# Autodesk Inventor assembly: FullApparatus
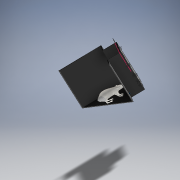
[picture p0: Inventor's stored thumbnail of the model, 180x180]
Saved by Autodesk Inventor 2020 (Build 240168000, 168)
## iProperties
Created: 2019-09-17
Part Number: FullApparatus
Document SubType Name: Assembly
Designer: Knowblesse
Author: Knowblesse
## Documents named in this file (5)
- C:\VCF\Lobster\Apparatus\FullApparatus.iam
- C:\VCF\Lobster\Apparatus\Arena\Main.ipt
- C:\VCF\Lobster\Apparatus\Robot\Motor_Panel.iam
- C:\VCF\Lobster\Apparatus\Arena\IRLight.ipt
- C:\VCF\Lobster\Apparatus\Visual\rat5su.ipt
## Components (4 placed, 4 different names)
1. Main:1 — 강체:1, 강체:2, 메이트:1, 메이트:2, 회전:1
2. Motor_Panel:1 [sub-assembly] — 강체:1
3. IRLight:1 — 강체:2
4. rat5su:1 — 회전:1
## Relationships (5: WeldJoint 2, Mate 2, RevoluteJoint 1)
- 강체:1 [WeldJoint]: Main:1 ↔ Motor_Panel:1
- 강체:2 [WeldJoint]: Main:1 ↔ IRLight:1
- 메이트:1 [Mate]: Main:1
- 메이트:2 [Mate]: Main:1
- 회전:1 [RevoluteJoint]: Main:1 ↔ rat5su:1
